# Autodesk Inventor assembly: Magazin
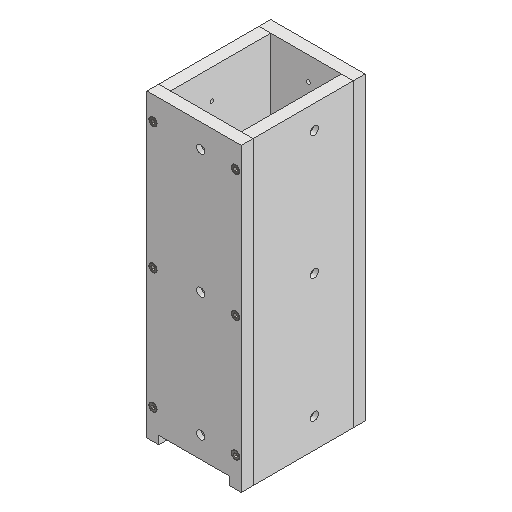
[picture p0: Inventor's stored thumbnail of the model, 512x512]
Saved by Autodesk Inventor 2025.1 (Build 291241000, 241)
## iProperties
Created: 2025-06-25
Part Number: Magazin
Document SubType Name: Assembly
Designer: Erik
Author: Erik
## Documents named in this file (6)
- C:\Users\Erik\Erik\Hochschule\3. Semester\CAD\CAD-Paspa\Useless Box\Eigene Bauteile\Fallmagazin\Magazin Wände\Magazin.iam
- C:\Users\Erik\Erik\Hochschule\3. Semester\CAD\CAD-Paspa\Useless Box\Eigene Bauteile\Fallmagazin\Magazin Wände\ER_Wand_1.ipt
- C:\Users\Erik\Erik\Hochschule\3. Semester\CAD\CAD-Paspa\Useless Box\Eigene Bauteile\Fallmagazin\Magazin Wände\ER_Wand_2.ipt
- C:\Users\Erik\Erik\Hochschule\3. Semester\CAD\CAD-Paspa\Useless Box\Eigene Bauteile\Fallmagazin\Magazin Wände\ER_Wand_3.ipt
- C:\Users\Erik\Erik\Hochschule\3. Semester\CAD\CAD-Paspa\Useless Box\Eigene Bauteile\Fallmagazin\Magazin Wände\ER_Wand_4.ipt
- C:\Users\Erik\Erik\Hochschule\3. Semester\CAD\CAD-Paspa\Useless Box\Standart Bauteile\DIN EN ISO 4762 - M4 x 16.ipt
## Components (16 placed, 5 different names)
1. ER_Wand_1:1 — Passend:1, Fluchtend:1, Fluchtend:2, Passend:2, Fluchtend:3, Fluchtend:4, Fluchtend:5, Fluchtend:6, Passend:3
2. ER_Wand_2:1 — Passend:2, Fluchtend:3, Fluchtend:4, Passend:4, Passend:5, Symmetrie:1, Einfügen:1, Einfügen:2, Einfügen:3
3. ER_Wand_3:1 — Passend:4, Passend:5, Fluchtend:7
4. ER_Wand_4:1 — Fluchtend:5, Fluchtend:6, Passend:3, Fluchtend:7, Symmetrie:1
5. DIN EN ISO 4762 - M4 x 16:5 — Einfügen:3
6. DIN EN ISO 4762 - M4 x 16:6 — Einfügen:2
7. DIN EN ISO 4762 - M4 x 16:7
8. DIN EN ISO 4762 - M4 x 16:8
9. DIN EN ISO 4762 - M4 x 16:9
10. DIN EN ISO 4762 - M4 x 16:10
11. DIN EN ISO 4762 - M4 x 16:11
12. DIN EN ISO 4762 - M4 x 16:12
13. DIN EN ISO 4762 - M4 x 16:1 — Einfügen:1
14. DIN EN ISO 4762 - M4 x 16:2
15. DIN EN ISO 4762 - M4 x 16:3
16. DIN EN ISO 4762 - M4 x 16:4
## Component patterns: (4 elements, first: DIN EN ISO 4762 - M4 x 16:1)
## Relationships (16: Flush 7, Mate 5, Insert 3, Symmetry 1)
- Passend:1 [Mate]: ER_Wand_1:1
- Fluchtend:1 [Flush]: ER_Wand_1:1
- Fluchtend:2 [Flush]: ER_Wand_1:1
- Passend:2 [Mate]: ER_Wand_1:1 ↔ ER_Wand_2:1
- Fluchtend:3 [Flush]: ER_Wand_1:1 ↔ ER_Wand_2:1
- Fluchtend:4 [Flush]: ER_Wand_1:1 ↔ ER_Wand_2:1
- Fluchtend:5 [Flush]: ER_Wand_1:1 ↔ ER_Wand_4:1
- Fluchtend:6 [Flush]: ER_Wand_1:1 ↔ ER_Wand_4:1
- Passend:3 [Mate]: ER_Wand_1:1 ↔ ER_Wand_4:1
- Passend:4 [Mate]: ER_Wand_2:1 ↔ ER_Wand_3:1
- Passend:5 [Mate] (-10 mm): ER_Wand_2:1 ↔ ER_Wand_3:1
- Fluchtend:7 [Flush]: ER_Wand_3:1 ↔ ER_Wand_4:1
- Symmetrie:1: ER_Wand_2:1 ↔ ER_Wand_4:1
- Einfügen:1 [Insert]: ER_Wand_2:1 ↔ DIN EN ISO 4762 - M4 x 16:1
- Einfügen:2 [Insert]: ER_Wand_2:1 ↔ DIN EN ISO 4762 - M4 x 16:6
- Einfügen:3 [Insert]: ER_Wand_2:1 ↔ DIN EN ISO 4762 - M4 x 16:5
